# Autodesk Inventor assembly: CanSat
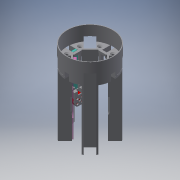
[picture p0: Inventor's stored thumbnail of the model, 180x180]
Saved by Autodesk Inventor 2018 (Build 220112000, 112)
## iProperties
Created: 2018-05-01
Part Number: CanSat
Document SubType Name: Assembly
Designer: suchanek
Author: suchanek
## Documents named in this file (11)
- C:\Users\sucha\programming\CanSat\CanSat2.0\Schematics\Model\CanSat.iam
- C:\Users\sucha\programming\CanSat\CanSat2.0\Schematics\Model\Hull_middle.ipt
- C:\Users\sucha\programming\CanSat\CanSat2.0\Schematics\Model\Hull_batt_pillar.ipt
- C:\Users\sucha\programming\CanSat\CanSat2.0\Schematics\Model\Circuit.ipt
- C:\Users\sucha\programming\CanSat\CanSat2.0\Schematics\Model\Motor_drivers.ipt
- C:\Users\sucha\programming\CanSat\CanSat2.0\Schematics\Model\Hull_main.ipt
- C:\Users\sucha\programming\CanSat\CanSat2.0\Schematics\Model\Circuit_center.ipt
- C:\Users\sucha\programming\CanSat\CanSat2.0\Schematics\Model\Arm.ipt
- C:\Users\sucha\programming\CanSat\CanSat2.0\Schematics\Model\Motor_holder.ipt
- C:\Users\sucha\programming\CanSat\CanSat2.0\Schematics\Model\Motor.ipt
- C:\Users\sucha\programming\CanSat\CanSat2.0\Schematics\Model\Rotor.ipt
## Components (13 placed, 10 different names)
1. Hull_middle:1 — Rotational:2, Angle:2, Rotational:3, Flush:2
2. Circuit:1 — Rotational:2, Angle:2, Angle:3
3. Motor_drivers:1 — Flush:1, Angle:4, Cylindrical:1
4. Hull_main:1 — Rotational:1, Angle:1, Rotational:3, Angle:3, Flush:1, Angle:4, Cylindrical:1, Rotational:4
5. Circuit_center:1 — Planar:1, Flush:2
6. Arm:1 — Rotational:4, Rigid:1
7. Motor_holder:1 — Rigid:1, Rigid:2
8. Motor:1 — Rigid:2, Rotational:5
9. Rotor:1 — Rotational:5
10. Hull_batt_pillar:1 — Rotational:1, Angle:1
11. Hull_batt_pillar:2 — Planar:1
12. Hull_batt_pillar:3
13. Hull_batt_pillar:4
## Component patterns: (4 elements, first: Hull_batt_pillar:1)
## Relationships (15: RevoluteJoint 5, Angle 4, Flush 2, WeldJoint 2, CylindricalJoint 1, PlanarJoint 1)
- Rotational:1 [RevoluteJoint]: Hull_main:1 ↔ Hull_batt_pillar:1
- Angle:1 (0 deg): Hull_main:1 ↔ Hull_batt_pillar:1
- Rotational:2 [RevoluteJoint]: Hull_middle:1 ↔ Circuit:1
- Angle:2 (0 deg): Hull_middle:1 ↔ Circuit:1
- Rotational:3 [RevoluteJoint]: Hull_middle:1 ↔ Hull_main:1
- Angle:3 (0 deg): Circuit:1 ↔ Hull_main:1
- Flush:1 (12 mm): Motor_drivers:1 ↔ Hull_main:1
- Angle:4 (0 deg): Motor_drivers:1 ↔ Hull_main:1
- Cylindrical:1: Motor_drivers:1 ↔ Hull_main:1
- Planar:1 (0.5 mm): Circuit_center:1 ↔ Hull_batt_pillar:2
- Flush:2 (3 mm): Hull_middle:1 ↔ Circuit_center:1
- Rotational:4 [RevoluteJoint] (-0.15 mm): Hull_main:1 ↔ Arm:1
- Rigid:1 [WeldJoint]: Arm:1 ↔ Motor_holder:1
- Rigid:2 [WeldJoint]: Motor_holder:1 ↔ Motor:1
- Rotational:5 [RevoluteJoint]: Motor:1 ↔ Rotor:1
